# Autodesk Inventor assembly: Grid_Of_Piers
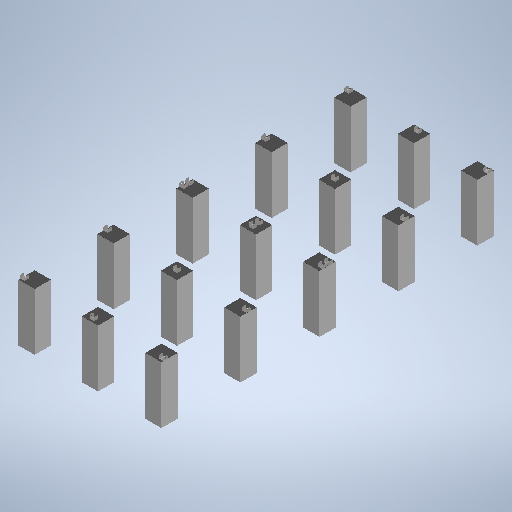
[picture p0: Inventor's stored thumbnail of the model, 512x512]
Saved by Autodesk Inventor 2025.1 (Build 291241020, 241B)
## iProperties
Created: 2024-08-07
Part Number: Grid_Of_Piers
Document SubType Name: Assembly
Designer: Tom
Author: Tom
## Documents named in this file (3)
- C:\Users\Tom\Documents\Inventor\Mobility\Additional_Building\Grid_Of_Piers.iam
- C:\Users\Tom\Documents\Inventor\Mobility\Additional_Building\Pier.iam
- C:\Users\Tom\Documents\Inventor\Mobility\Additional_Building\Saddle_Bracket.ipt
## Components (33 placed, 2 different names)
1. Saddle_Bracket:1 — Mate:1, Flush:1, Flush:2
2. Saddle_Bracket:2 — Mate:2, Flush:3, Mate:10
3. Saddle_Bracket:3 — Mate:3, Flush:5, Mate:11
4. Saddle_Bracket:4 — Mate:4, Flush:7, Mate:12
5. Saddle_Bracket:5 — Mate:5, Mate:6, Mate:7
6. Saddle_Bracket:6 — Mate:8, Mate:9, Mate:13
7. Saddle_Bracket:7 — Mate:14, Flush:8, Flush:9
8. Saddle_Bracket:8 — Mate:15, Flush:10, Mate:16
9. Saddle_Bracket:9 — Flush:11, Mate:17, Flush:12
10. Saddle_Bracket:10 — Mate:18, Mate:19, Flush:13
11. Saddle_Bracket:11 — Mate:20, Mate:21, Mate:22
12. Saddle_Bracket:12 — Mate:23, Flush:14, Mate:24
13. Saddle_Bracket:13 — Mate:25, Flush:15, Flush:18
14. Saddle_Bracket:14 — Mate:27, Mate:28, Flush:17
15. Saddle_Bracket:15 — Mate:30, Mate:31, Flush:16
16. Saddle_Bracket:16 — Mate:32, Mate:33, Flush:21
17. Saddle_Bracket:17 — Mate:35, Flush:19, Flush:20
18. Saddle_Bracket:18 — Mate:36, Flush:22, Flush:23
19. Pier:1 [sub-assembly] — Mate:1, Flush:1, Flush:2
20. Pier:2 [sub-assembly] — Mate:2, Flush:3, Mate:10
21. Pier:3 [sub-assembly] — Mate:3, Flush:5, Mate:11, Mate:14, Flush:8, Flush:9
22. Pier:4 [sub-assembly] — Mate:15, Flush:10, Mate:16
23. Pier:5 [sub-assembly] — Flush:11, Mate:17, Flush:12
24. Pier:6 [sub-assembly] — Mate:4, Flush:7, Mate:12
25. Pier:7 [sub-assembly] — Mate:5, Mate:6, Mate:7
26. Pier:8 [sub-assembly] — Mate:8, Mate:9, Mate:13, Mate:18, Mate:19, Flush:13
27. Pier:9 [sub-assembly] — Mate:20, Mate:21, Mate:22
28. Pier:10 [sub-assembly] — Mate:23, Flush:14, Mate:24
29. Pier:11 [sub-assembly] — Mate:25, Flush:15, Flush:18
30. Pier:12 [sub-assembly] — Mate:27, Mate:28, Flush:17
31. Pier:13 [sub-assembly] — Mate:30, Mate:31, Flush:16, Mate:36, Flush:22, Flush:23
32. Pier:14 [sub-assembly] — Mate:32, Mate:33, Flush:21
33. Pier:15 [sub-assembly] — Mate:35, Flush:19, Flush:20
## Component patterns: (15 elements, first: Pier:1)
## Relationships (54: Mate 33, Flush 21)
- Mate:1: Saddle_Bracket:1 ↔ Pier:1
- Flush:1 (-3.175 mm): Saddle_Bracket:1 ↔ Pier:1
- Flush:2 (41.275 mm): Saddle_Bracket:1 ↔ Pier:1
- Mate:2: Saddle_Bracket:2 ↔ Pier:2
- Flush:3 (-3.175 mm): Saddle_Bracket:2 ↔ Pier:2
- Mate:3: Saddle_Bracket:3 ↔ Pier:3
- Flush:5 (-3.175 mm): Saddle_Bracket:3 ↔ Pier:3
- Mate:4: Saddle_Bracket:4 ↔ Pier:6
- Flush:7 (41.275 mm): Saddle_Bracket:4 ↔ Pier:6
- Mate:5: Saddle_Bracket:5 ↔ Pier:7
- Mate:6: Saddle_Bracket:5 ↔ Pier:7
- Mate:7: Saddle_Bracket:5 ↔ Pier:7
- Mate:8: Saddle_Bracket:6 ↔ Pier:8
- Mate:9: Saddle_Bracket:6 ↔ Pier:8
- Mate:10: Saddle_Bracket:2 ↔ Pier:2
- Mate:11 (20.6375 mm): Saddle_Bracket:3 ↔ Pier:3
- Mate:12: Saddle_Bracket:4 ↔ Pier:6
- Mate:13 (20.6375 mm): Saddle_Bracket:6 ↔ Pier:8
- Mate:14: Saddle_Bracket:7 ↔ Pier:3
- Flush:8 (-3.175 mm): Saddle_Bracket:7 ↔ Pier:3
- Flush:9 (20.6375 mm): Saddle_Bracket:7 ↔ Pier:3
- Mate:15: Saddle_Bracket:8 ↔ Pier:4
- Flush:10 (-3.175 mm): Saddle_Bracket:8 ↔ Pier:4
- Mate:16: Saddle_Bracket:8 ↔ Pier:4
- Flush:11 (41.275 mm): Saddle_Bracket:9 ↔ Pier:5
- Mate:17: Saddle_Bracket:9 ↔ Pier:5
- Flush:12 (-3.175 mm): Saddle_Bracket:9 ↔ Pier:5
- Mate:18: Saddle_Bracket:10 ↔ Pier:8
- Mate:19: Saddle_Bracket:10 ↔ Pier:8
- Flush:13 (20.6375 mm): Saddle_Bracket:10 ↔ Pier:8
- Mate:20: Saddle_Bracket:11 ↔ Pier:9
- Mate:21: Saddle_Bracket:11 ↔ Pier:9
- Mate:22: Saddle_Bracket:11 ↔ Pier:9
- Mate:23: Saddle_Bracket:12 ↔ Pier:10
- Flush:14 (41.275 mm): Saddle_Bracket:12 ↔ Pier:10
- Mate:24: Saddle_Bracket:12 ↔ Pier:10
- Mate:25: Saddle_Bracket:13 ↔ Pier:11
- Flush:15 (41.275 mm): Saddle_Bracket:13 ↔ Pier:11
- Mate:27: Saddle_Bracket:14 ↔ Pier:12
- Mate:28: Saddle_Bracket:14 ↔ Pier:12
- Mate:30: Saddle_Bracket:15 ↔ Pier:13
- Mate:31 (20.6375 mm): Saddle_Bracket:15 ↔ Pier:13
- Flush:16 (-3.175 mm): Saddle_Bracket:15 ↔ Pier:13
- Flush:17 (-3.175 mm): Saddle_Bracket:14 ↔ Pier:12
- Flush:18 (-3.175 mm): Saddle_Bracket:13 ↔ Pier:11
- Mate:32: Saddle_Bracket:16 ↔ Pier:14
- Mate:33: Saddle_Bracket:16 ↔ Pier:14
- Mate:35: Saddle_Bracket:17 ↔ Pier:15
- Flush:19 (-3.175 mm): Saddle_Bracket:17 ↔ Pier:15
- Flush:20 (41.275 mm): Saddle_Bracket:17 ↔ Pier:15
- Flush:21 (-3.175 mm): Saddle_Bracket:16 ↔ Pier:14
- Mate:36: Saddle_Bracket:18 ↔ Pier:13
- Flush:22 (-3.175 mm): Saddle_Bracket:18 ↔ Pier:13
- Flush:23 (20.6375 mm): Saddle_Bracket:18 ↔ Pier:13
